# Autodesk Inventor assembly: Control Board Assembly
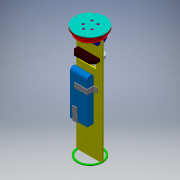
[picture p0: Inventor's stored thumbnail of the model, 180x180]
Saved by Autodesk Inventor 2016 (Build 200138000, 138)
## iProperties
Created: 2017-10-10
Part Number: Control Board Assembly
Document SubType Name: Assembly
Designer: Student
Author: Student
## Documents named in this file (17)
- C:\Users\Student\Documents\Derek Code and Projects\Autodesk\Control Board Assembly.iam
- C:\Users\Student\Documents\Derek Code and Projects\Autodesk\Control board Holder.ipt
- C:\Users\Student\Documents\Derek Code and Projects\Autodesk\Control Board.ipt
- C:\Users\Student\Documents\Derek Code and Projects\Autodesk\Control board Ring Holder.ipt
- C:\Users\Student\Documents\Derek Code and Projects\Autodesk\THE ACTUAL BACK O-RONG FITTING Connection to control board.ipt
- C:\Users\Student\Documents\Cylinder Clamp\Camera Mount.ipt
- C:\Users\Student\Documents\Derek Code and Projects\Autodesk\Camera.ipt
- C:\Users\Student\Documents\Derek Code and Projects\Autodesk\RPI.ipt
- C:\Users\Student\Documents\Derek Code and Projects\Autodesk\Arduino board with Sheild.ipt
- C:\Users\Student\Documents\Derek Code and Projects\Autodesk\Battery.ipt
- C:\Users\Student\Documents\Derek Code and Projects\Autodesk\Voltage Divider (Rough).ipt
- C:\Users\Student\Documents\Derek Code and Projects\Autodesk\Back Lens.ipt
- C:\Users\Student\Documents\Derek Code and Projects\Autodesk\Wire fitting End.ipt
- C:\Users\Student\Documents\Inventor\Content Center Files\R2016\en-US\BS 4183(7)\BS 4183 - M2.5 x 5(2) III.ipt
- C:\Users\Student\Documents\Inventor\Content Center Files\R2016\en-US\BS 4183(7)\BS 4183 - M3 x 5(2) III.ipt
- C:\Users\Student\Documents\Inventor\Content Center Files\R2016\en-US\BS 4183(7)\BS 4183 - M4 x 5(2) III.ipt
- C:\Users\Student\Documents\Derek Code and Projects\Autodesk\Battery Mount.ipt
## Components (41 placed, 16 different names)
1. Control board Holder:1 — Mate:36, Mate:37, Mate:38, Insert:13, Insert:14, Insert:15
2. Control board Holder:2 — Mate:34, Mate:35, Mate:39, Mate:40, Insert:10, Insert:11, Insert:12
3. Control Board:1 — Mate:29, Mate:30, Flush:1, Mate:31, Mate:32, Mate:33, Mate:34, Mate:35, Mate:36, Mate:37, Mate:41, Mate:42, Mate:43, Mate:46, Mate:47, Mate:48, Mate:49, Mate:50, Mate:51, Mate:52, Flush:2, Mate:53, Mate:54, Mate:55, Mate:56, Mate:57, Mate:58, Insert:8, Insert:9, Mate:72, Mate:73, Mate:74, Mate:75
4. Control board Ring Holder:1 — Mate:31, Mate:32, Mate:33
5. THE ACTUAL BACK O-RONG FITTING Connection to control board:1 — Mate:38, Mate:39, Mate:40, Mate:59, Mate:60, Mate:61
6. Camera Mount:1 — Mate:41, Mate:42, Mate:43, Mate:44, Mate:45, Insert:1, Insert:2, Insert:3, Insert:4
7. Camera:1 — Mate:44, Mate:45
8. RPI:1 — Mate:46, Mate:47, Mate:48, Flush:3
9. Arduino board with Sheild:1 — Mate:49, Mate:50, Mate:51, Insert:5, Insert:6, Insert:7
10. Battery:1 — Mate:52, Flush:2, Flush:3, Mate:76
11. Voltage Divider (Rough):1 — Mate:53, Mate:54, Mate:58
12. Voltage Divider (Rough):2 — Mate:55, Mate:56, Mate:57
13. Back Lens:1 — Mate:59, Mate:60, Mate:61, Mate:62, Mate:63, Mate:64, Mate:65, Mate:66, Mate:67, Mate:68, Mate:69, Mate:70, Mate:71, Insert:16, Insert:17, Insert:18, Insert:19, Insert:20, Insert:21
14. Wire fitting End:1 — Mate:64, Mate:65
15. Wire fitting End:2 — Mate:62, Mate:63
16. Wire fitting End:3 — Mate:68, Mate:69
17. Wire fitting End:4 — Mate:70, Mate:71
18. Wire fitting End:5 — Mate:66, Mate:67
19. BS 4183 Slotted Pan Head Machine Screw - Metric M2.5 x 5:1 — Insert:1
20. BS 4183 Slotted Pan Head Machine Screw - Metric M2.5 x 5:2 — Insert:2
21. BS 4183 Slotted Pan Head Machine Screw - Metric M2.5 x 5:3 — Insert:3
22. BS 4183 Slotted Pan Head Machine Screw - Metric M2.5 x 5:4 — Insert:4
23. BS 4183 Slotted Pan Head Machine Screw - Metric M3 x 5:1 — Insert:5
24. BS 4183 Slotted Pan Head Machine Screw - Metric M3 x 5:2 — Insert:6
25. BS 4183 Slotted Pan Head Machine Screw - Metric M3 x 5:3 — Insert:7
26. BS 4183 Slotted Pan Head Machine Screw - Metric M4 x 5:1 — Insert:8
27. BS 4183 Slotted Pan Head Machine Screw - Metric M4 x 5:2 — Insert:9
28. BS 4183 Slotted Pan Head Machine Screw - Metric M2.5 x 5:5 — Insert:10
29. BS 4183 Slotted Pan Head Machine Screw - Metric M2.5 x 5:6 — Insert:11
30. BS 4183 Slotted Pan Head Machine Screw - Metric M3 x 5:4 — Insert:12
31. BS 4183 Slotted Pan Head Machine Screw - Metric M2.5 x 5:7 — Insert:13
32. BS 4183 Slotted Pan Head Machine Screw - Metric M3 x 5:5 — Insert:14
33. BS 4183 Slotted Pan Head Machine Screw - Metric M2.5 x 5:8 — Insert:15
34. BS 4183 Slotted Pan Head Machine Screw - Metric M2.5 x 5:9 — Insert:16
35. BS 4183 Slotted Pan Head Machine Screw - Metric M2.5 x 5:10 — Insert:17
36. BS 4183 Slotted Pan Head Machine Screw - Metric M2.5 x 5:11 — Insert:18
37. BS 4183 Slotted Pan Head Machine Screw - Metric M2.5 x 5:12 — Insert:19
38. BS 4183 Slotted Pan Head Machine Screw - Metric M2.5 x 5:13 — Insert:20
39. BS 4183 Slotted Pan Head Machine Screw - Metric M2.5 x 5:14 — Insert:21
40. Battery Mount:1 — Mate:72, Mate:74
41. Battery Mount:3 — Mate:73, Mate:75, Mate:76
## Relationships (72: Mate 48, Insert 21, Flush 3)
- Mate:29: Control Board:1
- Mate:30: Control Board:1
- Flush:1: Control Board:1
- Mate:31: Control Board:1 ↔ Control board Ring Holder:1
- Mate:32: Control Board:1 ↔ Control board Ring Holder:1
- Mate:33: Control Board:1 ↔ Control board Ring Holder:1
- Mate:34: Control board Holder:2 ↔ Control Board:1
- Mate:35: Control board Holder:2 ↔ Control Board:1
- Mate:36: Control board Holder:1 ↔ Control Board:1
- Mate:37: Control board Holder:1 ↔ Control Board:1
- Mate:38: Control board Holder:1 ↔ THE ACTUAL BACK O-RONG FITTING Connection to control board:1
- Mate:39: Control board Holder:2 ↔ THE ACTUAL BACK O-RONG FITTING Connection to control board:1
- Mate:40: Control board Holder:2 ↔ THE ACTUAL BACK O-RONG FITTING Connection to control board:1
- Mate:41: Control Board:1 ↔ Camera Mount:1
- Mate:42: Control Board:1 ↔ Camera Mount:1
- Mate:43: Control Board:1 ↔ Camera Mount:1
- Mate:44: Camera Mount:1 ↔ Camera:1
- Mate:45: Camera Mount:1 ↔ Camera:1
- Mate:46: Control Board:1 ↔ RPI:1
- Mate:47: Control Board:1 ↔ RPI:1
- Mate:48: Control Board:1 ↔ RPI:1
- Mate:49: Control Board:1 ↔ Arduino board with Sheild:1
- Mate:50: Control Board:1 ↔ Arduino board with Sheild:1
- Mate:51: Control Board:1 ↔ Arduino board with Sheild:1
- Mate:52: Control Board:1 ↔ Battery:1
- Flush:2: Control Board:1 ↔ Battery:1
- Flush:3: RPI:1 ↔ Battery:1
- Mate:53: Control Board:1 ↔ Voltage Divider (Rough):1
- Mate:54: Control Board:1 ↔ Voltage Divider (Rough):1
- Mate:55: Control Board:1 ↔ Voltage Divider (Rough):2
- Mate:56: Control Board:1 ↔ Voltage Divider (Rough):2
- Mate:57: Control Board:1 ↔ Voltage Divider (Rough):2
- Mate:58: Control Board:1 ↔ Voltage Divider (Rough):1
- Mate:59: THE ACTUAL BACK O-RONG FITTING Connection to control board:1 ↔ Back Lens:1
- Mate:60: THE ACTUAL BACK O-RONG FITTING Connection to control board:1 ↔ Back Lens:1
- Mate:61: THE ACTUAL BACK O-RONG FITTING Connection to control board:1 ↔ Back Lens:1
- Mate:62: Back Lens:1 ↔ Wire fitting End:2
- Mate:63: Back Lens:1 ↔ Wire fitting End:2
- Mate:64: Back Lens:1 ↔ Wire fitting End:1
- Mate:65: Back Lens:1 ↔ Wire fitting End:1
- Mate:66: Back Lens:1 ↔ Wire fitting End:5
- Mate:67: Back Lens:1 ↔ Wire fitting End:5
- Mate:68: Back Lens:1 ↔ Wire fitting End:3
- Mate:69: Back Lens:1 ↔ Wire fitting End:3
- Mate:70: Back Lens:1 ↔ Wire fitting End:4
- Mate:71: Back Lens:1 ↔ Wire fitting End:4
- Insert:1: Camera Mount:1 ↔ BS 4183 Slotted Pan Head Machine Screw - Metric M2.5 x 5:1
- Insert:2: Camera Mount:1 ↔ BS 4183 Slotted Pan Head Machine Screw - Metric M2.5 x 5:2
- Insert:3: Camera Mount:1 ↔ BS 4183 Slotted Pan Head Machine Screw - Metric M2.5 x 5:3
- Insert:4: Camera Mount:1 ↔ BS 4183 Slotted Pan Head Machine Screw - Metric M2.5 x 5:4
- Insert:5: Arduino board with Sheild:1 ↔ BS 4183 Slotted Pan Head Machine Screw - Metric M3 x 5:1
- Insert:6: Arduino board with Sheild:1 ↔ BS 4183 Slotted Pan Head Machine Screw - Metric M3 x 5:2
- Insert:7: Arduino board with Sheild:1 ↔ BS 4183 Slotted Pan Head Machine Screw - Metric M3 x 5:3
- Insert:8: Control Board:1 ↔ BS 4183 Slotted Pan Head Machine Screw - Metric M4 x 5:1
- Insert:9: Control Board:1 ↔ BS 4183 Slotted Pan Head Machine Screw - Metric M4 x 5:2
- Insert:10: Control board Holder:2 ↔ BS 4183 Slotted Pan Head Machine Screw - Metric M2.5 x 5:5
- Insert:11: Control board Holder:2 ↔ BS 4183 Slotted Pan Head Machine Screw - Metric M2.5 x 5:6
- Insert:12: Control board Holder:2 ↔ BS 4183 Slotted Pan Head Machine Screw - Metric M3 x 5:4
- Insert:13: Control board Holder:1 ↔ BS 4183 Slotted Pan Head Machine Screw - Metric M2.5 x 5:7
- Insert:14: Control board Holder:1 ↔ BS 4183 Slotted Pan Head Machine Screw - Metric M3 x 5:5
- Insert:15: Control board Holder:1 ↔ BS 4183 Slotted Pan Head Machine Screw - Metric M2.5 x 5:8
- Insert:16: Back Lens:1 ↔ BS 4183 Slotted Pan Head Machine Screw - Metric M2.5 x 5:9
- Insert:17: Back Lens:1 ↔ BS 4183 Slotted Pan Head Machine Screw - Metric M2.5 x 5:10
- Insert:18: Back Lens:1 ↔ BS 4183 Slotted Pan Head Machine Screw - Metric M2.5 x 5:11
- Insert:19: Back Lens:1 ↔ BS 4183 Slotted Pan Head Machine Screw - Metric M2.5 x 5:12
- Insert:20: Back Lens:1 ↔ BS 4183 Slotted Pan Head Machine Screw - Metric M2.5 x 5:13
- Insert:21: Back Lens:1 ↔ BS 4183 Slotted Pan Head Machine Screw - Metric M2.5 x 5:14
- Mate:72: Control Board:1 ↔ Battery Mount:1
- Mate:73: Control Board:1 ↔ Battery Mount:3
- Mate:74: Control Board:1 ↔ Battery Mount:1
- Mate:75: Control Board:1 ↔ Battery Mount:3
- Mate:76: Battery:1 ↔ Battery Mount:3
